# Autodesk Inventor assembly: Assembly
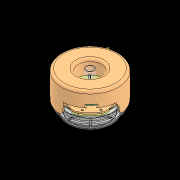
[picture p0: Inventor's stored thumbnail of the model, 180x180]
Saved by Autodesk Inventor 2022 (Build 260153000, 153)
## iProperties
Created: 2021-10-30
Part Number: Assembly
Document SubType Name: Assembly
Designer: alber
Author: alber
## Documents named in this file (12)
- C:\Users\alber\Desktop\Files\Università\V ANNO ACCADEMICO\Capstone Project\Qura-ECC-Pump-Tester\design\Assembly.iam
- C:\Users\alber\Desktop\Files\Università\V ANNO ACCADEMICO\Capstone Project\Qura-ECC-Pump-Tester\design\Housing.ipt
- C:\Users\alber\Desktop\Files\Università\V ANNO ACCADEMICO\Capstone Project\Qura-ECC-Pump-Tester\design\Pump.ipt
- C:\Users\alber\Desktop\Files\Università\V ANNO ACCADEMICO\Capstone Project\Qura-ECC-Pump-Tester\design\Sensor.ipt
- C:\Users\alber\Desktop\Files\Università\V ANNO ACCADEMICO\Capstone Project\Qura-ECC-Pump-Tester\design\Driver.ipt
- C:\Users\alber\Desktop\Files\Università\V ANNO ACCADEMICO\Capstone Project\Qura-ECC-Pump-Tester\design\Driver_lock.ipt
- C:\Users\alber\Desktop\Files\Università\V ANNO ACCADEMICO\Capstone Project\Qura-ECC-Pump-Tester\design\VSlider.ipt
- C:\Users\alber\Desktop\Files\Università\V ANNO ACCADEMICO\Capstone Project\Qura-ECC-Pump-Tester\design\sliderr.ipt
- C:\Users\alber\Desktop\Files\Università\V ANNO ACCADEMICO\Capstone Project\Qura-ECC-Pump-Tester\design\nema17.ipt
- C:\Users\alber\Desktop\Files\Università\V ANNO ACCADEMICO\Capstone Project\Qura-ECC-Pump-Tester\pcb\qura_pump_pcb_model.ipt
- C:\Users\alber\Desktop\Files\Università\V ANNO ACCADEMICO\Capstone Project\Qura-ECC-Pump-Tester\design\Assembly\Design Accelerator\Spur Gears2.iam
- C:\Users\alber\Desktop\Files\Università\V ANNO ACCADEMICO\Capstone Project\Qura-ECC-Pump-Tester\design\Case.ipt
## Components (16 placed, 11 different names)
1. Sensor:1 — Mate:4, Cylindrical:12
2. Sensor:2 — Mate:2, Cylindrical:10
3. Sensor:3 — Mate:5, Cylindrical:9
4. Sensor:4 — Mate:7, Cylindrical:14
5. Sensor:5 — Mate:6, Cylindrical:13
6. Sensor:6 — Mate:3, Cylindrical:11
7. Pump:1 — Cylindrical:8, Cylindrical:16, Cylindrical:17
8. Housing:1 — Mate:2, Mate:3, Mate:4, Mate:5, Mate:6, Mate:7, Cylindrical:9, Cylindrical:10, Cylindrical:11, Cylindrical:12, Cylindrical:13, Cylindrical:14, Cylindrical:16, Insert:1
9. Driver:1 — Cylindrical:8, Mate:8, Flush:1, Mate:9, Mate:15, Mate:16
10. Driver_lock:1 — Mate:8, Flush:1, Mate:9, Flush:3, Mate:10
11. VSlider:1 — Flush:3, Mate:10, Mate:11, Flush:4
12. sliderr:1 — Mate:11, Flush:4, Mate:12, Mate:13, Mate:14
13. nema17:1 — Mate:12, Mate:13, Mate:14, Cylindrical:15
14. qura_pump_pcb_model:1 — Insert:1
15. Spur Gears:1 [sub-assembly] — Cylindrical:15, Mate:15, Mate:16
16. Case:1 — Cylindrical:17
## Relationships (29: Mate 15, CylindricalJoint 10, Flush 3, Insert 1)
- Mate:2: Sensor:2 ↔ Housing:1
- Mate:3: Sensor:6 ↔ Housing:1
- Mate:4: Sensor:1 ↔ Housing:1
- Mate:5: Sensor:3 ↔ Housing:1
- Mate:6: Sensor:5 ↔ Housing:1
- Mate:7: Sensor:4 ↔ Housing:1
- Cylindrical:8: Pump:1 ↔ Driver:1
- Mate:8: Driver:1 ↔ Driver_lock:1
- Flush:1: Driver:1 ↔ Driver_lock:1
- Mate:9: Driver:1 ↔ Driver_lock:1
- Flush:3: Driver_lock:1 ↔ VSlider:1
- Mate:10 (1 mm): Driver_lock:1 ↔ VSlider:1
- Mate:11: VSlider:1 ↔ sliderr:1
- Flush:4: VSlider:1 ↔ sliderr:1
- Mate:12: sliderr:1 ↔ nema17:1
- Mate:13 (0.5 mm): sliderr:1 ↔ nema17:1
- Mate:14 (0.5 mm): sliderr:1 ↔ nema17:1
- Cylindrical:9: Sensor:3 ↔ Housing:1
- Cylindrical:10: Sensor:2 ↔ Housing:1
- Cylindrical:11: Sensor:6 ↔ Housing:1
- Cylindrical:12: Sensor:1 ↔ Housing:1
- Cylindrical:13: Sensor:5 ↔ Housing:1
- Cylindrical:14: Sensor:4 ↔ Housing:1
- Cylindrical:15: nema17:1 ↔ Spur Gears:1
- Mate:15: Driver:1 ↔ Spur Gears:1
- Mate:16: Driver:1 ↔ Spur Gears:1
- Cylindrical:16: Pump:1 ↔ Housing:1
- Insert:1: Housing:1 ↔ qura_pump_pcb_model:1
- Cylindrical:17: Pump:1 ↔ Case:1
